# Autodesk Inventor assembly: EngineAssemblyNEW
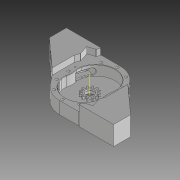
[picture p0: Inventor's stored thumbnail of the model, 180x180]
Saved by Autodesk Inventor 2020 (Build 240168000, 168)
## iProperties
Created: 2021-02-15
Part Number: EngineAssemblyNEW
Document SubType Name: Assembly
Designer: DDeGo
Author: DDeGo
## Documents named in this file (4)
- C:\Users\DDeGo\Documents\Drew\Projects\AirWankelEngine\cad\EngineAssemblyNEW.iam
- C:\Users\DDeGo\Documents\Drew\Projects\AirWankelEngine\cad\housingNEW.ipt
- C:\Users\DDeGo\Documents\Drew\Projects\AirWankelEngine\cad\housingValveNEW.ipt
- C:\Users\DDeGo\Documents\Drew\Projects\AirWankelEngine\cad\ValveFlapper.ipt
## Components (4 placed, 3 different names)
1. housingNEW:1 — Mate:1, Mate:2, Mate:3, Mate:4, Mate:5, Mate:6, Mate:7, Mate:8
2. housingValveNEW:1 — Mate:1, Mate:5, Mate:6
3. ValveFlapper:1 — Mate:7, Mate:8
4. housingValveNEW:2 — Mate:2, Mate:3, Mate:4
## Relationships (8: Mate 8)
- Mate:1: housingNEW:1 ↔ housingValveNEW:1
- Mate:2: housingNEW:1 ↔ housingValveNEW:2
- Mate:3: housingNEW:1 ↔ housingValveNEW:2
- Mate:4: housingNEW:1 ↔ housingValveNEW:2
- Mate:5: housingNEW:1 ↔ housingValveNEW:1
- Mate:6: housingNEW:1 ↔ housingValveNEW:1
- Mate:7: housingNEW:1 ↔ ValveFlapper:1
- Mate:8 (0.2 mm): housingNEW:1 ↔ ValveFlapper:1
